# Autodesk Inventor assembly: 85824-HUB
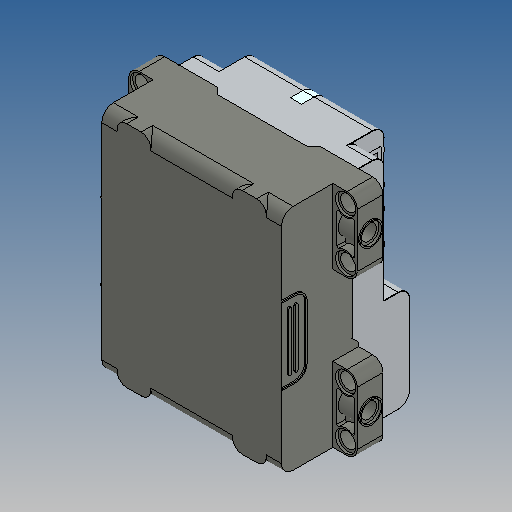
[picture p0: Inventor's stored thumbnail of the model, 512x512]
Saved by Autodesk Inventor 2025 (Build 290162010, 162A)
## iProperties
Created: 2024-11-22
Part Number: 85824-HUB
Material: Generisch
Description: NOT SPECIFIED
Document SubType Name: Assembly
Designer: hp.muther
Author: hp.muther
Revision Number: 1LAST_VERSION
## Documents named in this file (4)
- D:\Inventor\Projekte\Muther\LEGO Technic\LEGO Pieces\85824 - HUB.iam
- D:\Inventor\Projekte\Muther\LEGO Technic\LEGO Pieces\_Einzelteile zu Baugruppen\85824-01.ipt
- D:\Inventor\Projekte\Muther\LEGO Technic\LEGO Pieces\_Einzelteile zu Baugruppen\85824-02.ipt
- D:\Inventor\Projekte\Muther\LEGO Technic\LEGO Pieces\_Einzelteile zu Baugruppen\85824-03.ipt
## Components (6 placed, 3 different names)
1. 85824-01:1 — Passend:3, Fluchtend:2, Fluchtend:3
2. 85824-02:1 — Passend:3, Fluchtend:2, Fluchtend:3
3. 85824-03:1
4. 85824-03:2
5. 85824-03:3
6. 85824-03:4
## Relationships (3: Flush 2, Mate 1)
- Passend:3 [Mate]: 85824-01:1 ↔ 85824-02:1
- Fluchtend:2 [Flush]: 85824-01:1 ↔ 85824-02:1
- Fluchtend:3 [Flush]: 85824-01:1 ↔ 85824-02:1
